# Autodesk Inventor assembly: Final
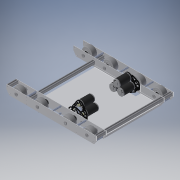
[picture p0: Inventor's stored thumbnail of the model, 180x180]
Saved by Autodesk Inventor 2016 (Build 200138000, 138)
## iProperties
Created: 2017-01-19
Part Number: Final
Document SubType Name: Assembly
Designer: Kyle
Author: Kyle
## Documents named in this file (10)
- E:\1073CAD\Robot2017\DriveTrain\Final.iam
- E:\1073CAD\Robot2017\DriveTrain\OutsidePlate.ipt
- E:\1073CAD\Robot2017\DriveTrain\Individual Parts\Mock 8020 28.25in.ipt
- E:\1073CAD\Robot2017\DriveTrain\InsidePlate.ipt
- E:\1073CAD\Robot2017\DriveTrain\Individual Parts\3.625Churro.ipt
- E:\1073CAD\Robot2017\DriveTrain\Individual Parts\SinglePulley.iam
- E:\1073CAD\Robot2017\DriveTrain\Individual Parts\DoublePulley.iam
- E:\1073CAD\Robot2017\DriveTrain\Individual Parts\DoublePulleyGearbox.iam
- E:\1073CAD\Robot2017\DriveTrain\Individual Parts\Mock 8020 3.375in.ipt
- E:\1073CAD\Robot2017\DriveTrain\BellyPan.ipt
## Components (32 placed, 9 different names)
1. OutsidePlate:1
2. Mock 8020 28.25in:1
3. Mock 8020 28.25in:2
4. InsidePlate:1 — Flush:1
5. 3.625Churro:1
6. 3.625Churro:2
7. 3.625Churro:3
8. 3.625Churro:4
9. 3.625Churro:5
10. 3.625Churro:6
11. 3.625Churro:7
12. 3.625Churro:9
13. OutsidePlate:2
14. 3.625Churro:10
15. 3.625Churro:11
16. 3.625Churro:12
17. 3.625Churro:13
18. 3.625Churro:14
19. 3.625Churro:15
20. 3.625Churro:16
21. 3.625Churro:18
22. InsidePlate:2 — Mate:1
23. SinglePulley:1 [sub-assembly]
24. SinglePulley:2 [sub-assembly]
25. SinglePulley:3 [sub-assembly]
26. SinglePulley:4 [sub-assembly]
27. DoublePulley:1 [sub-assembly]
28. DoublePulley:2 [sub-assembly]
29. DoublePulleyGearbox:1 [sub-assembly]
30. DoublePulleyGearbox:2 [sub-assembly]
31. Mock 8020 3.375in:1
32. BellyPan:1 — Mate:1, Flush:1
## Relationships (2: Mate 1, Flush 1)
- Mate:1: InsidePlate:2 ↔ BellyPan:1
- Flush:1: InsidePlate:1 ↔ BellyPan:1
